# Autodesk Inventor assembly: EyasSay_Ensamblaje
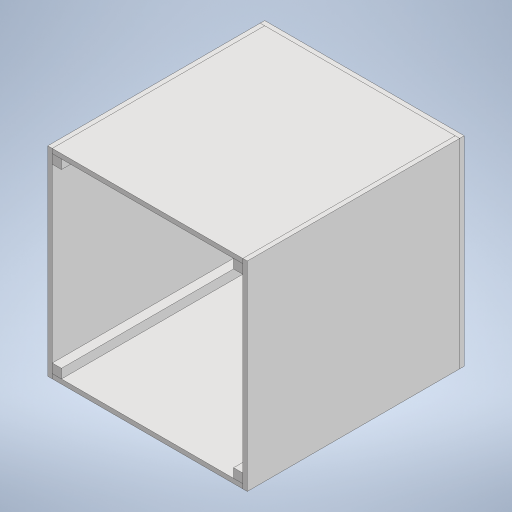
[picture p0: Inventor's stored thumbnail of the model, 512x512]
Saved by Autodesk Inventor 2024 (Build 280153000, 153)
## iProperties
Created: 2023-06-26
Part Number: EyasSay_Ensamblaje
Document SubType Name: Assembly
Designer: Personal
Author: Personal
## Documents named in this file (11)
- D:\Personal\Documents\GitHub\TDG_ReactionWheelsUnloading\Inventor\EyasSat_medicionesReales\EyasSay_Ensamblaje.iam
- D:\Personal\Documents\GitHub\TDG_ReactionWheelsUnloading\Inventor\EyasSat_medicionesReales\Acrilico_Bottom.ipt
- D:\Personal\Documents\GitHub\TDG_ReactionWheelsUnloading\Inventor\EyasSat_medicionesReales\AcrilicoX.ipt
- D:\Personal\Documents\GitHub\TDG_ReactionWheelsUnloading\Inventor\EyasSat_medicionesReales\AcrilicoX_MIR.ipt
- D:\Personal\Documents\GitHub\TDG_ReactionWheelsUnloading\Inventor\EyasSat_medicionesReales\AcrilicoY.ipt
- D:\Personal\Documents\GitHub\TDG_ReactionWheelsUnloading\Inventor\EyasSat_medicionesReales\AcrilicoY_MIR.ipt
- D:\Personal\Documents\GitHub\TDG_ReactionWheelsUnloading\Inventor\EyasSat_medicionesReales\BarraVertical.ipt
- D:\Personal\Documents\GitHub\TDG_ReactionWheelsUnloading\Inventor\EyasSat_medicionesReales\BarraVertical_MIR.ipt
- D:\Personal\Documents\GitHub\TDG_ReactionWheelsUnloading\Inventor\EyasSat_medicionesReales\BarraVertical_MIR1.ipt
- D:\Personal\Documents\GitHub\TDG_ReactionWheelsUnloading\Inventor\EyasSat_medicionesReales\BarraVertical_MIR_MIR.ipt
- D:\Personal\Documents\GitHub\TDG_ReactionWheelsUnloading\Inventor\EyasSat_medicionesReales\PCB_COM_BAT.ipt
## Components (10 placed, 10 different names)
1. Acrilico_Bottom:1 — Coincidencia:1, Coincidencia:2, Coincidencia:3, Coincidencia:4, Nivelación:1, Nivelación:2, Coincidencia:5, Nivelación:3, Nivelación:4, Nivelación:5, Nivelación:6, Nivelación:7, Coincidencia:8, Nivelación:8, Nivelación:9, Nivelación:10, Coincidencia:9, Nivelación:12, Coincidencia:12
2. AcrilicoX:1 — Coincidencia:4, Nivelación:1, Nivelación:2, Coincidencia:7, Coincidencia:10
3. AcrilicoX_MIR:1 — Coincidencia:5, Nivelación:3, Nivelación:4, Coincidencia:6
4. AcrilicoY:1 — Nivelación:5, Nivelación:6, Coincidencia:6, Nivelación:7
5. AcrilicoY_MIR:1 — Coincidencia:7, Coincidencia:8, Nivelación:8, Coincidencia:11, Nivelación:11
6. BarraVertical:1 — Nivelación:9, Nivelación:10, Coincidencia:9, Coincidencia:10, Coincidencia:11, Nivelación:11
7. BarraVertical_MIR:1
8. BarraVertical_MIR1:1
9. BarraVertical_MIR_MIR:1
10. PCB_COM_BAT:1 — Nivelación:12, Coincidencia:12
## Relationships (24: Mate 12, Flush 12)
- Coincidencia:1 [Mate] (-106 mm): Acrilico_Bottom:1
- Coincidencia:2 [Mate] (-97.5 mm): Acrilico_Bottom:1
- Coincidencia:3 [Mate] (-97.5 mm): Acrilico_Bottom:1
- Coincidencia:4 [Mate]: Acrilico_Bottom:1 ↔ AcrilicoX:1
- Nivelación:1 [Flush]: Acrilico_Bottom:1 ↔ AcrilicoX:1
- Nivelación:2 [Flush]: Acrilico_Bottom:1 ↔ AcrilicoX:1
- Coincidencia:5 [Mate]: Acrilico_Bottom:1 ↔ AcrilicoX_MIR:1
- Nivelación:3 [Flush]: Acrilico_Bottom:1 ↔ AcrilicoX_MIR:1
- Nivelación:4 [Flush]: Acrilico_Bottom:1 ↔ AcrilicoX_MIR:1
- Nivelación:5 [Flush]: Acrilico_Bottom:1 ↔ AcrilicoY:1
- Nivelación:6 [Flush]: Acrilico_Bottom:1 ↔ AcrilicoY:1
- Coincidencia:6 [Mate]: AcrilicoX_MIR:1 ↔ AcrilicoY:1
- Nivelación:7 [Flush]: Acrilico_Bottom:1 ↔ AcrilicoY:1
- Coincidencia:7 [Mate]: AcrilicoX:1 ↔ AcrilicoY_MIR:1
- Coincidencia:8 [Mate]: Acrilico_Bottom:1 ↔ AcrilicoY_MIR:1
- Nivelación:8 [Flush]: Acrilico_Bottom:1 ↔ AcrilicoY_MIR:1
- Nivelación:9 [Flush]: Acrilico_Bottom:1 ↔ BarraVertical:1
- Nivelación:10 [Flush]: Acrilico_Bottom:1 ↔ BarraVertical:1
- Coincidencia:9 [Mate]: Acrilico_Bottom:1 ↔ BarraVertical:1
- Coincidencia:10 [Mate]: AcrilicoX:1 ↔ BarraVertical:1
- Coincidencia:11 [Mate]: AcrilicoY_MIR:1 ↔ BarraVertical:1
- Nivelación:11 [Flush]: AcrilicoY_MIR:1 ↔ BarraVertical:1
- Nivelación:12 [Flush]: Acrilico_Bottom:1 ↔ PCB_COM_BAT:1
- Coincidencia:12 [Mate]: Acrilico_Bottom:1 ↔ PCB_COM_BAT:1
